# Autodesk Inventor assembly: wheel_set
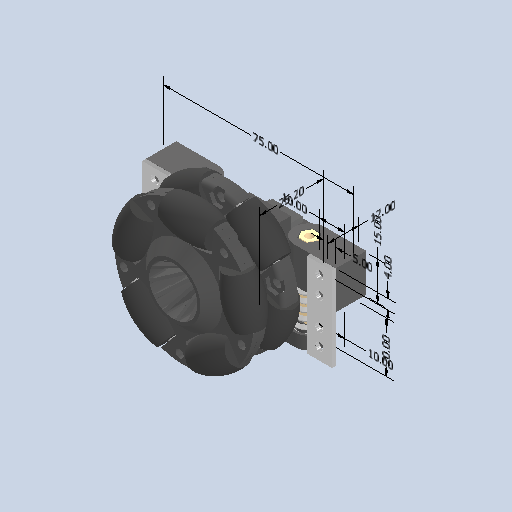
[picture p0: Inventor's stored thumbnail of the model, 512x512]
Saved by Autodesk Inventor 2024.1 (Build 281209000, 209)
## iProperties
Created: 2024-12-19
Part Number: wheel_set
Document SubType Name: Assembly
Designer: hibik
Author: hibik
## Documents named in this file (8)
- C:\Users\hibik\Documents\Robomech\RESCUE\ORCA\hard\omni_wheel\Assy_omni_wheel.iam
- C:\Users\hibik\Documents\Robomech\RESCUE\ORCA\hard\omni_wheel\Assy_motor.iam
- C:\Users\hibik\Documents\Robomech\RESCUE\ORCA\hard\omni_wheel\Assy_wheel.iam
- C:\Users\hibik\Documents\Robomech\RESCUE\ORCA\hard\std_parts\bearing_3_6_2.5.ipt
- C:\Users\hibik\Documents\Robomech\RESCUE\ORCA\hard\std_parts\spring_pi10_23.ipt
- C:\Users\hibik\Documents\Robomech\RESCUE\ORCA\hard\omni_wheel\spacer.ipt
- C:\Users\hibik\Documents\Robomech\RESCUE\ORCA\hard\omni_wheel\wheel_setter.ipt
- C:\Users\hibik\Documents\Robomech\RESCUE\ORCA\hard\omni_wheel\wheel_setter_plate.ipt
## Components (13 placed, 7 different names)
1. Assy_motor:1 [sub-assembly] — 挿入:1, 挿入:2, 挿入:3, 挿入:4, 挿入:5, 挿入:6, 挿入:7, 挿入:8, 挿入:9, 角度:1, 角度:2
2. Assy_wheel:1 [sub-assembly] — 挿入:5
3. bearing_3_6_2.5:1 — 挿入:1
4. bearing_3_6_2.5:2 — 挿入:2
5. bearing_3_6_2.5:3 — 挿入:3
6. bearing_3_6_2.5:4 — 挿入:4
7. spring_pi10_23:1 — 挿入:7
8. spring_pi10_23:2 — 挿入:6
9. spacer:1 — 挿入:9, 角度:1
10. spacer:2 — 挿入:8, 角度:2, 挿入:10, 角度:4
11. wheel_setter:1 — 挿入:10, 角度:4, 挿入:11, 挿入:12, 挿入:13, 挿入:14
12. wheel_setter_plate:1 — 挿入:11, 挿入:12
13. wheel_setter_plate:2 — 挿入:13, 挿入:14
## Relationships (17: Insert 14, Angle 3)
- 挿入:1 [Insert]: Assy_motor:1 ↔ bearing_3_6_2.5:1
- 挿入:2 [Insert]: Assy_motor:1 ↔ bearing_3_6_2.5:2
- 挿入:3 [Insert]: Assy_motor:1 ↔ bearing_3_6_2.5:3
- 挿入:4 [Insert]: Assy_motor:1 ↔ bearing_3_6_2.5:4
- 挿入:5 [Insert]: Assy_motor:1 ↔ Assy_wheel:1
- 挿入:6 [Insert]: Assy_motor:1 ↔ spring_pi10_23:2
- 挿入:7 [Insert]: Assy_motor:1 ↔ spring_pi10_23:1
- 挿入:8 [Insert]: Assy_motor:1 ↔ spacer:2
- 挿入:9 [Insert]: Assy_motor:1 ↔ spacer:1
- 角度:1 [Angle] (0 deg): Assy_motor:1 ↔ spacer:1
- 角度:2 [Angle] (0 deg): Assy_motor:1 ↔ spacer:2
- 挿入:10 [Insert] (0.01 mm): spacer:2 ↔ wheel_setter:1
- 角度:4 [Angle] (180 deg): spacer:2 ↔ wheel_setter:1
- 挿入:11 [Insert]: wheel_setter:1 ↔ wheel_setter_plate:1
- 挿入:12 [Insert]: wheel_setter:1 ↔ wheel_setter_plate:1
- 挿入:13 [Insert]: wheel_setter:1 ↔ wheel_setter_plate:2
- 挿入:14 [Insert]: wheel_setter:1 ↔ wheel_setter_plate:2
